# Autodesk Inventor assembly: SPE48V2 Roldana Acrilico
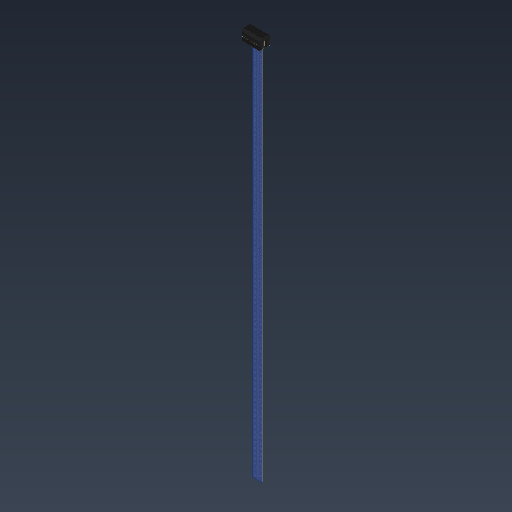
[picture p0: Inventor's stored thumbnail of the model, 512x512]
Saved by Autodesk Inventor 2021.2 (Build 252289000, 289)
## iProperties
Created: 2026-09-01
Part Number: SPE48V2 Roldana Acrilico
Document SubType Name: Assembly
Designer: nelso
Mass: 602.524 g
Surface Area: 3556.14 cm^2
Volume: 516.501 cm^3
Density: 1.16655 g/cm^3
Author: nelso
## Documents named in this file (7)
- C:\Users\nelso\Documents\Escritorio\Soporte-Paciente-Espinografia\Workspace\SPE48V2 Roldana Acrilico.iam
- C:\Users\nelso\Documents\Escritorio\Soporte-Paciente-Espinografia\Workspace\SP46V1 Felpa Roldana.ipt
- C:\Users\nelso\Documents\Escritorio\Soporte-Paciente-Espinografia\Workspace\SP50V2 Acrilico Roldana.ipt
- C:\Users\nelso\Documents\Escritorio\Soporte-Paciente-Espinografia\Workspace\SP53V1 Acrilico superior.ipt
- C:\Users\nelso\Documents\Escritorio\Soporte-Paciente-Espinografia\Workspace\SP45V2 Plastico Roldana.ipt
- C:\Users\nelso\Documents\Escritorio\Soporte-Paciente-Espinografia\Workspace\DIN555-5M4X0.8I.ipt
- C:\Users\nelso\Documents\Escritorio\Soporte-Paciente-Espinografia\Workspace\DIN7991M4X0.8L16C.ipt
## Components (9 placed, 6 different names)
1. SP45V2 Plastico Roldana:1 — Mate:4, Mate:5, Mate:6, Flush:1, Flush:2, Mate:7, Mate:8, Mate:9, Mate:10, Mate:13, Mate:14, Mate:15, Flush:5, Mate:16, Mate:17
2. SP50V2 Acrilico Roldana:1 — Mate:1, Mate:2, Mate:3, Mate:4, Mate:11, Mate:12
3. SP53V1 Acrilico superior:1 — Mate:1, Mate:2, Mate:3, Mate:5, Mate:6, Flush:3, Flush:4
4. DIN555-5M4X0.8I:1 — Mate:9, Mate:10
5. DIN555-5M4X0.8I:2 — Mate:7, Mate:8
6. DIN7991M4X0.8L16C:1 — Mate:11, Flush:3
7. DIN7991M4X0.8L16C:2 — Mate:12, Flush:4
8. SP46V1 Felpa Roldana:1 — Mate:13, Flush:5, Mate:16
9. SP46V1 Felpa Roldana:2 — Mate:14, Mate:15, Mate:17
## Relationships (22: Mate 17, Flush 5)
- Mate:1: SP50V2 Acrilico Roldana:1 ↔ SP53V1 Acrilico superior:1
- Mate:2: SP50V2 Acrilico Roldana:1 ↔ SP53V1 Acrilico superior:1
- Mate:3: SP50V2 Acrilico Roldana:1 ↔ SP53V1 Acrilico superior:1
- Mate:4: SP45V2 Plastico Roldana:1 ↔ SP50V2 Acrilico Roldana:1
- Mate:5: SP45V2 Plastico Roldana:1 ↔ SP53V1 Acrilico superior:1
- Mate:6: SP45V2 Plastico Roldana:1 ↔ SP53V1 Acrilico superior:1
- Flush:1: SP45V2 Plastico Roldana:1
- Flush:2: SP45V2 Plastico Roldana:1
- Mate:7: SP45V2 Plastico Roldana:1 ↔ DIN555-5M4X0.8I:2
- Mate:8: SP45V2 Plastico Roldana:1 ↔ DIN555-5M4X0.8I:2
- Mate:9: SP45V2 Plastico Roldana:1 ↔ DIN555-5M4X0.8I:1
- Mate:10: SP45V2 Plastico Roldana:1 ↔ DIN555-5M4X0.8I:1
- Mate:11: SP50V2 Acrilico Roldana:1 ↔ DIN7991M4X0.8L16C:1
- Mate:12: SP50V2 Acrilico Roldana:1 ↔ DIN7991M4X0.8L16C:2
- Flush:3: SP53V1 Acrilico superior:1 ↔ DIN7991M4X0.8L16C:1
- Flush:4: SP53V1 Acrilico superior:1 ↔ DIN7991M4X0.8L16C:2
- Mate:13: SP45V2 Plastico Roldana:1 ↔ SP46V1 Felpa Roldana:1
- Mate:14: SP45V2 Plastico Roldana:1 ↔ SP46V1 Felpa Roldana:2
- Mate:15: SP45V2 Plastico Roldana:1 ↔ SP46V1 Felpa Roldana:2
- Flush:5: SP45V2 Plastico Roldana:1 ↔ SP46V1 Felpa Roldana:1
- Mate:16: SP45V2 Plastico Roldana:1 ↔ SP46V1 Felpa Roldana:1
- Mate:17: SP45V2 Plastico Roldana:1 ↔ SP46V1 Felpa Roldana:2
